# Autodesk Inventor assembly: 3_finger_gripper_b
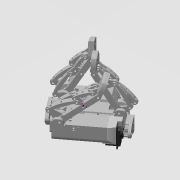
[picture p0: Inventor's stored thumbnail of the model, 180x180]
Saved by Autodesk Inventor 2016 (Build 200138000, 138)
## iProperties
Created: 2015-01-03
Part Number: 3_finger_gripper_b
Document SubType Name: Assembly
Designer: 4ndreas
Mass: 285.047 g
Surface Area: 1445.43 cm^2
Volume: 240.209 cm^3
Density: 1.18666 g/cm^3
Author: 4ndreas
## Documents named in this file (6)
- C:\Users\4ndreas\Documents\Inventor\RobotARM v2\Gripper V1\3_finger_gripper_b.iam
- C:\Users\4ndreas\Documents\Inventor\RobotARM v2\Gripper V1\Finger_clean.iam
- C:\Users\4ndreas\Documents\Inventor\RobotARM v2\Gripper V1\Finger_L.iam
- C:\Users\4ndreas\Documents\Inventor\RobotARM v2\Gripper V1\Finger_L1.iam
- C:\Users\4ndreas\Documents\Inventor\RobotARM v2\Gripper V1\kipprad.ipt
- C:\Users\4ndreas\Documents\Inventor\RobotARM v2\Gripper V1\Stirnzahnrad13.ipt
## Components (5 placed, 5 different names)
1. Finger_clean:1 [sub-assembly] — Passend:28, Passend:69, Passend:72, Passend:73, Passend:78, Passend:79, Passend:83, Winkel:2
2. Finger_L:1 [sub-assembly] — Passend:75, Fluchtend:1, Fluchtend:3, Drehung:1, Winkel:2, Passend:84, Passend:85
3. Finger_L1:1 [sub-assembly] — Passend:28, Passend:74, Fluchtend:1, Fluchtend:3, Drehung:1
4. kipprad:1 — Passend:82, Passend:83
5. Stirnzahnrad1:1 — Passend:84, Passend:85
## Relationships (21: Mate 17, Flush 2, RelateRotation 1, Angle 1)
- Passend:28 [Mate]: Finger_clean:1 ↔ Finger_L1:1
- Passend:69 [Mate]: Finger_clean:1
- Passend:71 [Mate]
- Passend:72 [Mate]: Finger_clean:1
- Passend:73 [Mate]: Finger_clean:1
- Passend:74 [Mate]: Finger_L1:1
- Passend:75 [Mate]: Finger_L:1
- Passend:76 [Mate]
- Passend:77 [Mate]
- Passend:78 [Mate]: Finger_clean:1
- Passend:79 [Mate]: Finger_clean:1
- Passend:80 [Mate]
- Passend:81 [Mate]
- Fluchtend:1 [Flush]: Finger_L:1 ↔ Finger_L1:1
- Passend:82 [Mate]: kipprad:1
- Passend:83 [Mate]: Finger_clean:1 ↔ kipprad:1
- Fluchtend:3 [Flush]: Finger_L:1 ↔ Finger_L1:1
- Drehung:1 [RelateRotation] (1 ul): Finger_L:1 ↔ Finger_L1:1
- Winkel:2 [Angle] (145 deg): Finger_clean:1 ↔ Finger_L:1
- Passend:84 [Mate]: Finger_L:1 ↔ Stirnzahnrad1:1
- Passend:85 [Mate] (1 mm): Finger_L:1 ↔ Stirnzahnrad1:1
